# Autodesk Inventor assembly: Suberstructure
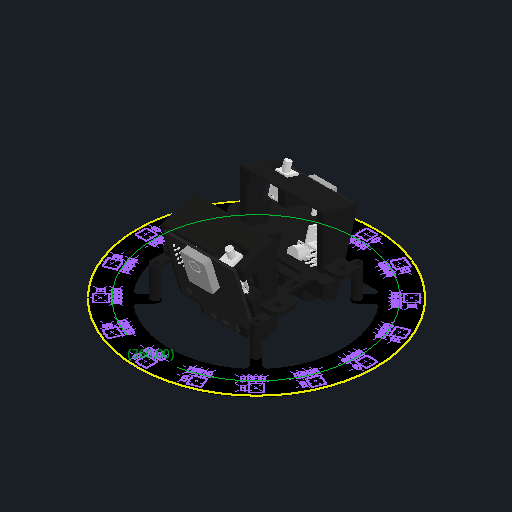
[picture p0: Inventor's stored thumbnail of the model, 512x512]
Saved by Autodesk Inventor 2023 (Build 270158000, 158)
## iProperties
Created: 2023-05-12
Part Number: Suberstructure
Document SubType Name: Assembly
Designer: Elias Braun
Author: Elias Braun
## Documents named in this file (5)
- C:\Users\Elias Braun\Nextcloud2\RoboCup2023\Suberstructure.iam
- C:\Users\Elias Braun\Nextcloud2\RoboCup2023\PCB\InfraredPCB.ipt
- C:\Users\Elias Braun\Nextcloud2\RoboCup2023\Connectors\IRSPacer-Pixy-(FT).ipt
- C:\Users\Elias Braun\Nextcloud2\RoboCup2023\Miscellaneous\HandleHolder_V2.ipt
- C:\Users\Elias Braun\Nextcloud2\RoboCup2023\Cam\CamComplete.iam
## Components (8 placed, 4 different names)
1. InfraredPCB:1 — Mate:1, Mate:2, Mate:3, Mate:4, Mate:5, Mate:6, Mate:7, Mate:8
2. IRSPacer-Pixy-(FT):1 — Mate:2, Mate:7
3. IRSPacer-Pixy-(FT):2 — Mate:4, Mate:5, Mate:20
4. IRSPacer-Pixy-(FT):3 — Mate:1, Mate:8, Mate:18, Mate:19
5. IRSPacer-Pixy-(FT):4 — Mate:3, Mate:6
6. HandleHolder_V2:1 — Mate:14, Mate:15, Mate:16, Mate:17, Mate:18, Mate:19, Mate:20, Mate:21, Mate:22
7. CamComplete:1 [sub-assembly] — Mate:15, Mate:16, Mate:17
8. CamComplete:2 [sub-assembly] — Mate:14, Mate:21, Mate:22
## Relationships (17: Mate 17)
- Mate:1: InfraredPCB:1 ↔ IRSPacer-Pixy-(FT):3
- Mate:2: InfraredPCB:1 ↔ IRSPacer-Pixy-(FT):1
- Mate:3: InfraredPCB:1 ↔ IRSPacer-Pixy-(FT):4
- Mate:4: InfraredPCB:1 ↔ IRSPacer-Pixy-(FT):2
- Mate:5: InfraredPCB:1 ↔ IRSPacer-Pixy-(FT):2
- Mate:6: InfraredPCB:1 ↔ IRSPacer-Pixy-(FT):4
- Mate:7: InfraredPCB:1 ↔ IRSPacer-Pixy-(FT):1
- Mate:8: InfraredPCB:1 ↔ IRSPacer-Pixy-(FT):3
- Mate:14: HandleHolder_V2:1 ↔ CamComplete:2
- Mate:15: HandleHolder_V2:1 ↔ CamComplete:1
- Mate:16: HandleHolder_V2:1 ↔ CamComplete:1
- Mate:17: HandleHolder_V2:1 ↔ CamComplete:1
- Mate:18: IRSPacer-Pixy-(FT):3 ↔ HandleHolder_V2:1
- Mate:19: IRSPacer-Pixy-(FT):3 ↔ HandleHolder_V2:1
- Mate:20: IRSPacer-Pixy-(FT):2 ↔ HandleHolder_V2:1
- Mate:21: HandleHolder_V2:1 ↔ CamComplete:2
- Mate:22: HandleHolder_V2:1 ↔ CamComplete:2
